# Autodesk Inventor assembly: derive_rod_v7
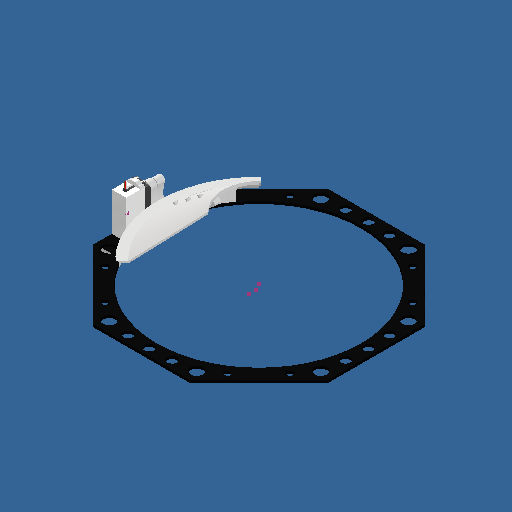
[picture p0: Inventor's stored thumbnail of the model, 512x512]
Saved by Autodesk Inventor 2026.2 (Build 302298000, 298)
## iProperties
Created: 2026-01-13
Part Number: derive_rod_v7
Document SubType Name: Assembly
Designer: Thoma
Author: Thoma
## Documents named in this file (12)
- C:\Users\Thoma\OneDrive\Desktop\dir\telescope_cover\cover\main.iam
- C:\Users\Thoma\OneDrive\Desktop\dir\telescope_cover\telescope\version_3\Telescope_End.ipt
- C:\Users\Thoma\OneDrive\Desktop\dir\telescope_cover\cover\Cover_Upper_v3.ipt
- C:\Users\Thoma\OneDrive\Desktop\dir\telescope_cover\servo\DSS-M15S Servo.ipt
- C:\Users\Thoma\OneDrive\Desktop\dir\telescope_cover\cover\rod_v10.ipt
- C:\Users\Thoma\OneDrive\Desktop\dir\telescope_cover\cover\Base_Plate_bottom.ipt
- C:\Users\Thoma\OneDrive\Desktop\dir\telescope_cover\cover\4mm_screw.ipt
- C:\Users\Thoma\OneDrive\Desktop\dir\telescope_cover\cover\6mm_washer_1mm.ipt
- C:\Users\Thoma\OneDrive\Desktop\dir\telescope_cover\cover\pawn.ipt
- C:\Users\Thoma\OneDrive\Desktop\dir\telescope_cover\cover\base_plate_v5.ipt
- C:\Users\Thoma\OneDrive\Desktop\dir\telescope_cover\cover\4mm_washer_1mm.ipt
- C:\Users\Thoma\OneDrive\Desktop\dir\telescope_cover\telescope\version_3\4mm_0.5_Screw.ipt
## Components (26 placed, 11 different names)
1. Telescope_End:1 — Flush:1, Mate:24, Mate:47, Mate:48, Mate:49
2. Cover_Upper_v3:1 — Mate:15, Mate:16, Tangent:1, Mate:79, Mate:80, Mate:82, Mate:83, Mate:84
3. DSS-M15S Servo:1 — Flush:1, Mate:17, Mate:18, Angle:3, Mate:50, Mate:51, Mate:56, Angle:7
4. rod_v10:1 — Mate:15, Mate:16, Mate:17, Mate:18, Mate:57, Mate:73, Mate:74, Mate:75, Mate:76, Mate:77, Mate:78, Angle:11, Mate:81, Angle:12, Angle:13, Angle:14
5. Base_Plate_bottom:1 — Mate:24, Mate:25, Mate:26, Angle:1, Mate:52, Flush:3, Flush:4, Mate:53, Angle:5, Mate:54, Mate:55, Angle:6
6. 4mm_screw:1 — Mate:25, Mate:26, Angle:1
7. 6mm_washer_1mm:1 — Mate:30, Mate:66, Mate:67, Mate:68
8. 4mm_screw:2 — Mate:30, Angle:3, Mate:68
9. 4mm_screw:3 — Mate:34, Mate:71, Mate:72, Angle:10
10. 4mm_screw:4 — Mate:42, Mate:64, Mate:65, Angle:9
11. 4mm_screw:5 — Mate:38, Mate:60, Mate:61, Angle:8
12. 6mm_washer_1mm:2 — Mate:38, Mate:58, Mate:59, Mate:60, Mate:61
13. 6mm_washer_1mm:3 — Mate:42, Mate:62, Mate:63, Mate:64, Mate:65
14. 6mm_washer_1mm:4 — Mate:34, Mate:69, Mate:70, Mate:71, Mate:72
15. base_plate_v5:1 — Mate:43, Flush:2, Mate:44, Mate:45, Mate:46, Angle:4, Mate:47, Mate:48, Mate:49, Mate:50, Mate:51, Flush:3, Flush:4, Mate:58, Mate:59, Angle:8, Mate:62, Mate:63, Angle:9, Mate:66, Mate:67, Mate:69, Mate:70, Angle:10, Angle:14
16. pawn:1 — Mate:43, Flush:2, Mate:44
17. 4mm_screw:6 — Mate:45, Mate:46, Angle:4
18. 4mm_screw:7 — Mate:54, Mate:55, Angle:6
19. 4mm_screw:8 — Mate:52, Mate:53, Angle:5
20. 4mm_screw:9 — Mate:56, Mate:57, Angle:7
21. 4mm_0.5_Screw:1 — Mate:81, Mate:82, Angle:12
22. 4mm_0.5_Screw:2 — Mate:83, Mate:84, Angle:13
23. 4mm_0.5_Screw:3 — Mate:79, Mate:80, Angle:11
24. 4mm_washer_1mm:2 — Mate:73, Mate:74, Tangent:1
25. 4mm_washer_1mm:3 — Mate:77, Mate:78
26. 4mm_washer_1mm:4 — Mate:75, Mate:76
## Relationships (71: Mate 53, Angle 13, Flush 4, Tangent 1)
- Flush:1 (2.5 mm): Telescope_End:1 ↔ DSS-M15S Servo:1
- Mate:15: Cover_Upper_v3:1 ↔ rod_v10:1
- Mate:16: Cover_Upper_v3:1 ↔ rod_v10:1
- Mate:17: DSS-M15S Servo:1 ↔ rod_v10:1
- Mate:18: DSS-M15S Servo:1 ↔ rod_v10:1
- Mate:24: Telescope_End:1 ↔ Base_Plate_bottom:1
- Mate:25: Base_Plate_bottom:1 ↔ 4mm_screw:1
- Mate:26: Base_Plate_bottom:1 ↔ 4mm_screw:1
- Angle:1 (0 deg): Base_Plate_bottom:1 ↔ 4mm_screw:1
- Mate:30: 6mm_washer_1mm:1 ↔ 4mm_screw:2
- Angle:3 (0 deg): DSS-M15S Servo:1 ↔ 4mm_screw:2
- Mate:34: 4mm_screw:3 ↔ 6mm_washer_1mm:4
- Mate:38: 4mm_screw:5 ↔ 6mm_washer_1mm:2
- Mate:42: 4mm_screw:4 ↔ 6mm_washer_1mm:3
- Mate:43: base_plate_v5:1 ↔ pawn:1
- Flush:2 (3.5 mm): base_plate_v5:1 ↔ pawn:1
- Mate:44: base_plate_v5:1 ↔ pawn:1
- Mate:45: base_plate_v5:1 ↔ 4mm_screw:6
- Mate:46: base_plate_v5:1 ↔ 4mm_screw:6
- Angle:4 (0 deg): base_plate_v5:1 ↔ 4mm_screw:6
- Mate:47: Telescope_End:1 ↔ base_plate_v5:1
- Mate:48: Telescope_End:1 ↔ base_plate_v5:1
- Mate:49: Telescope_End:1 ↔ base_plate_v5:1
- Mate:50 (1.1 mm): DSS-M15S Servo:1 ↔ base_plate_v5:1
- Mate:51: DSS-M15S Servo:1 ↔ base_plate_v5:1
- Mate:52: Base_Plate_bottom:1 ↔ 4mm_screw:8
- Flush:3: Base_Plate_bottom:1 ↔ base_plate_v5:1
- Flush:4: Base_Plate_bottom:1 ↔ base_plate_v5:1
- Mate:53: Base_Plate_bottom:1 ↔ 4mm_screw:8
- Angle:5 (0 deg): Base_Plate_bottom:1 ↔ 4mm_screw:8
- Mate:54: Base_Plate_bottom:1 ↔ 4mm_screw:7
- Mate:55: Base_Plate_bottom:1 ↔ 4mm_screw:7
- Angle:6 (0 deg): Base_Plate_bottom:1 ↔ 4mm_screw:7
- Mate:56: DSS-M15S Servo:1 ↔ 4mm_screw:9
- Mate:57: rod_v10:1 ↔ 4mm_screw:9
- Angle:7 (0 deg): DSS-M15S Servo:1 ↔ 4mm_screw:9
- Mate:58: 6mm_washer_1mm:2 ↔ base_plate_v5:1
- Mate:59: 6mm_washer_1mm:2 ↔ base_plate_v5:1
- Mate:60: 4mm_screw:5 ↔ 6mm_washer_1mm:2
- Mate:61: 4mm_screw:5 ↔ 6mm_washer_1mm:2
- Angle:8 (0 deg): 4mm_screw:5 ↔ base_plate_v5:1
- Mate:62: 6mm_washer_1mm:3 ↔ base_plate_v5:1
- Mate:63: 6mm_washer_1mm:3 ↔ base_plate_v5:1
- Mate:64: 4mm_screw:4 ↔ 6mm_washer_1mm:3
- Mate:65: 4mm_screw:4 ↔ 6mm_washer_1mm:3
- Angle:9 (0 deg): 4mm_screw:4 ↔ base_plate_v5:1
- Mate:66: 6mm_washer_1mm:1 ↔ base_plate_v5:1
- Mate:67: 6mm_washer_1mm:1 ↔ base_plate_v5:1
- Mate:68: 6mm_washer_1mm:1 ↔ 4mm_screw:2
- Mate:69: 6mm_washer_1mm:4 ↔ base_plate_v5:1
- Mate:70: 6mm_washer_1mm:4 ↔ base_plate_v5:1
- Mate:71: 4mm_screw:3 ↔ 6mm_washer_1mm:4
- Mate:72: 4mm_screw:3 ↔ 6mm_washer_1mm:4
- Angle:10 (0 deg): 4mm_screw:3 ↔ base_plate_v5:1
- Mate:73: rod_v10:1 ↔ 4mm_washer_1mm:2
- Mate:74: rod_v10:1 ↔ 4mm_washer_1mm:2
- Mate:75: rod_v10:1 ↔ 4mm_washer_1mm:4
- Mate:76: rod_v10:1 ↔ 4mm_washer_1mm:4
- Mate:77: rod_v10:1 ↔ 4mm_washer_1mm:3
- Mate:78: rod_v10:1 ↔ 4mm_washer_1mm:3
- Tangent:1: Cover_Upper_v3:1 ↔ 4mm_washer_1mm:2
- Mate:79: Cover_Upper_v3:1 ↔ 4mm_0.5_Screw:3
- Mate:80: Cover_Upper_v3:1 ↔ 4mm_0.5_Screw:3
- Angle:11 (0 deg): rod_v10:1 ↔ 4mm_0.5_Screw:3
- Mate:81: rod_v10:1 ↔ 4mm_0.5_Screw:1
- Mate:82: Cover_Upper_v3:1 ↔ 4mm_0.5_Screw:1
- Angle:12 (0 deg): rod_v10:1 ↔ 4mm_0.5_Screw:1
- Mate:83: Cover_Upper_v3:1 ↔ 4mm_0.5_Screw:2
- Mate:84: Cover_Upper_v3:1 ↔ 4mm_0.5_Screw:2
- Angle:13 (0 deg): rod_v10:1 ↔ 4mm_0.5_Screw:2
- Angle:14 (233 deg): rod_v10:1 ↔ base_plate_v5:1
